# Autodesk Inventor assembly: Assembly
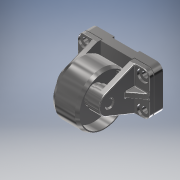
[picture p0: Inventor's stored thumbnail of the model, 180x180]
Saved by Autodesk Inventor 2019 (Build 230136000, 136)
## iProperties
Created: 2021-06-13
Part Number: Assembly
Document SubType Name: Assembly
Designer: joelm
Author: joelm
## Documents named in this file (5)
- C:\Users\joelm\OneDrive\Desktop\4.1\Manufacturing Tech\DieSets2\Assembly.iam
- C:\Users\joelm\OneDrive\Desktop\4.1\Manufacturing Tech\DieSets2\axle.ipt
- C:\Users\joelm\OneDrive\Desktop\4.1\Manufacturing Tech\DieSets2\axleSupport.ipt
- C:\Users\joelm\OneDrive\Desktop\4.1\Manufacturing Tech\DieSets2\topPlate.ipt
- C:\Users\joelm\OneDrive\Desktop\4.1\Manufacturing Tech\DieSets2\wheel.ipt
## Components (5 placed, 4 different names)
1. axle:1 — Mate:1, Flush:1, Mate:2, Flush:2
2. axleSupport:1 — Mate:2, Mate:4, Mate:6, Mate:7
3. topPlate:1 — Mate:4, Mate:5, Mate:6, Mate:7, Mate:8, Flush:2
4. wheel:1 — Mate:1, Flush:1, Mate:3
5. axleSupport:2 — Mate:3, Mate:5, Mate:8
## Relationships (10: Mate 8, Flush 2)
- Mate:1: axle:1 ↔ wheel:1
- Flush:1 (-20 mm): axle:1 ↔ wheel:1
- Mate:2: axle:1 ↔ axleSupport:1
- Mate:3: wheel:1 ↔ axleSupport:2
- Mate:4: axleSupport:1 ↔ topPlate:1
- Mate:5: topPlate:1 ↔ axleSupport:2
- Mate:6: axleSupport:1 ↔ topPlate:1
- Mate:7: axleSupport:1 ↔ topPlate:1
- Mate:8: topPlate:1 ↔ axleSupport:2
- Flush:2 (29 mm): axle:1 ↔ topPlate:1
